# Autodesk Inventor assembly: Bird_wing_assembly_V2_with_shoulder
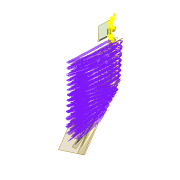
[picture p0: Inventor's stored thumbnail of the model, 180x180]
Saved by Autodesk Inventor 2022 (Build 260153000, 153)
## iProperties
Created: 2022-04-28
Part Number: Bird_wing_assembly_V2_with_shoulder
Document SubType Name: Assembly
Designer: dell
Mass: 4396.41 g
Surface Area: 10173.4 cm^2
Volume: 3712.61 cm^3
Author: dell
## Documents named in this file (4)
- D:\xxxx\Uni\Part IV\MECHENG_700\Part_IV_project_CAD\Bird_skeleton_prototypes\Wing_drone_V1\Bird_wing_V2\Bird_wing_assembly_V2_with_shoulder.iam
- D:\xxxx\Uni\Part IV\MECHENG_700\Part_IV_project_CAD\Bird_skeleton_prototypes\Wing_drone_V1\Bird_wing_V2\Bird_wing_assembly_V2.iam
- D:\xxxx\Uni\Part IV\MECHENG_700\Part_IV_project_CAD\Bird_skeleton_prototypes\Wing_drone_V1\Bird_wing_V2\Primary_hinge_guide_pulley_fix.ipt
- D:\xxxx\Uni\Part IV\MECHENG_700\Part_IV_project_CAD\Bird_skeleton_prototypes\Wing_drone_V1\Bird_wing_V2\Wing_shoulder\Shoulder_support_assembly_without_mount.iam
## Components (3 placed, 3 different names)
1. Bird_wing_assembly_V2:1 [sub-assembly] — Mate:1, Mate:2, Angle:1
2. Primary_hinge_guide_pulley_fix:1
3. Shoulder_support_assembly_without_mount:1 [sub-assembly] — Mate:1, Mate:2, Angle:1
## Relationships (3: Mate 2, Angle 1)
- Mate:1: Bird_wing_assembly_V2:1 ↔ Shoulder_support_assembly_without_mount:1
- Mate:2: Bird_wing_assembly_V2:1 ↔ Shoulder_support_assembly_without_mount:1
- Angle:1 (0 deg): Bird_wing_assembly_V2:1 ↔ Shoulder_support_assembly_without_mount:1
